# Autodesk Inventor assembly: Cover V3 Assembly
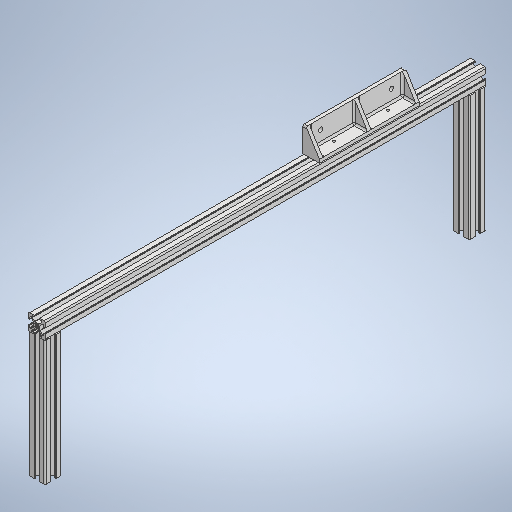
[picture p0: Inventor's stored thumbnail of the model, 512x512]
Saved by Autodesk Inventor 2025 (Build 290162000, 162)
## iProperties
Created: 2025-06-17
Part Number: Cover V3 Assembly
Document SubType Name: Assembly
Designer: mumin
Author: mumin
## Documents named in this file (4)
- C:\GitHub\In-situ-monitoring-of-powder-bed-fusion-additive-manufacturing\system_development\Orichalcum\v0.3\Cover v3 Assembly\Cover V3 Assembly.iam
- C:\GitHub\In-situ-monitoring-of-powder-bed-fusion-additive-manufacturing\system_development\Orichalcum\v0.3\Cover v3 Assembly\2020 Legs (150mm).ipt
- C:\GitHub\In-situ-monitoring-of-powder-bed-fusion-additive-manufacturing\system_development\Orichalcum\v0.3\Cover v3 Assembly\2020 LV-GVS Beam (530).ipt
- C:\GitHub\In-situ-monitoring-of-powder-bed-fusion-additive-manufacturing\system_development\Orichalcum\v0.3\Cover v3 Assembly\LV_Bracket_2.ipt
## Components (4 placed, 3 different names)
1. 2020 Legs (150mm):1 — Flush:1, Flush:2, Mate:1
2. 2020 Legs (150mm):2 — Mate:2, Flush:3, Flush:4
3. 2020 LV-GVS Beam (530):1 — Flush:1, Flush:2, Mate:1, Mate:2, Flush:3, Flush:4, Mate:3, Flush:5
4. LV_Bracket_2:1 — Mate:3, Flush:5
## Relationships (8: Flush 5, Mate 3)
- Flush:1: 2020 Legs (150mm):1 ↔ 2020 LV-GVS Beam (530):1
- Flush:2: 2020 Legs (150mm):1 ↔ 2020 LV-GVS Beam (530):1
- Mate:1: 2020 Legs (150mm):1 ↔ 2020 LV-GVS Beam (530):1
- Mate:2: 2020 Legs (150mm):2 ↔ 2020 LV-GVS Beam (530):1
- Flush:3: 2020 Legs (150mm):2 ↔ 2020 LV-GVS Beam (530):1
- Flush:4: 2020 Legs (150mm):2 ↔ 2020 LV-GVS Beam (530):1
- Mate:3: 2020 LV-GVS Beam (530):1 ↔ LV_Bracket_2:1
- Flush:5: 2020 LV-GVS Beam (530):1 ↔ LV_Bracket_2:1
